# Autodesk Inventor assembly: Assembly3(Rocker arm Sub Assembly)
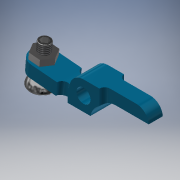
[picture p0: Inventor's stored thumbnail of the model, 180x180]
Saved by Autodesk Inventor 2018 (Build 220112000, 112)
## iProperties
Created: 2023-04-15
Part Number: Assembly3(Rocker arm Sub Assembly)
Document SubType Name: Assembly
Designer: Habib Mohamed
Author: Habib Mohamed
## Documents named in this file (4)
- D:\Inventor\My projects\Rotary Engine\Assembly\Assembly3(Rocker arm Sub Assembly).iam
- D:\Inventor\My projects\Rotary Engine\Component 28 (Rocker Arm Linkage).ipt
- D:\Inventor\My projects\Rotary Engine\Component 47(Rocker Arm).ipt
- C:\Users\Habib Mohamed\Documents\Inventor\Content Center Files\R2018\en-US\DIN EN 24 036(2)\DIN EN 24 036 - M3.ipt
## Components (3 placed, 3 different names)
1. Component 28 (Rocker Arm Linkage):1 — Mate:1, Flush:1, Mate:2
2. Component 47(Rocker Arm):1 — Mate:1, Flush:1, Mate:3
3. DIN EN 24036 M3:1 — Mate:2, Mate:3
## Relationships (4: Mate 3, Flush 1)
- Mate:1: Component 28 (Rocker Arm Linkage):1 ↔ Component 47(Rocker Arm):1
- Flush:1 (-4.5 mm): Component 28 (Rocker Arm Linkage):1 ↔ Component 47(Rocker Arm):1
- Mate:2: Component 28 (Rocker Arm Linkage):1 ↔ DIN EN 24036 M3:1
- Mate:3: Component 47(Rocker Arm):1 ↔ DIN EN 24036 M3:1
